# Autodesk Inventor assembly: 3組合1
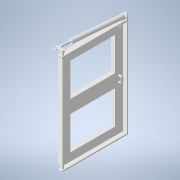
[picture p0: Inventor's stored thumbnail of the model, 180x180]
Saved by Autodesk Inventor 2020 (Build 240168000, 168)
## iProperties
Created: 2021-04-09
Part Number: 3組合1
Document SubType Name: Assembly
Designer: Sugar
Author: Sugar
## Documents named in this file (9)
- E:\github\cd2021\零件圖\stage2\3組合1.iam
- E:\github\cd2021\零件圖\stage2\3零件2.ipt
- E:\github\cd2021\零件圖\stage2\3零件3.ipt
- E:\github\cd2021\零件圖\stage2\3零件4.ipt
- E:\github\cd2021\零件圖\stage2\3零件5.ipt
- E:\github\cd2021\零件圖\stage2\3零件6.ipt
- E:\github\cd2021\零件圖\stage2\3零件7.ipt
- E:\github\cd2021\零件圖\stage2\3零件8.ipt
- E:\github\cd2021\零件圖\stage2\3零件10.ipt
## Components (8 placed, 8 different names)
1. 3零件5:1 — 插入:1, 貼合:4, 相切:1, 相切:2, 角度:2
2. 3零件6:1 — 貼合:1, 角度:1, 插入:5
3. 3零件7:2 — 插入:6
4. 3零件8:1 — 插入:1, 插入:2, 貼合:2
5. 3零件10:1 — 插入:2
6. 3零件2:1 — 插入:4, 插入:5, 插入:6, 相切:2
7. 3零件3:1 — 插入:3, 插入:4, 角度:1, 角度:2
8. 3零件4:1 — 插入:3, 貼合:4, 相切:1
## Relationships (14: Insert 6, Mate 4, Tangent 2, Angle 2)
- 插入:1 [Insert]: 3零件5:1 ↔ 3零件8:1
- 插入:2 [Insert]: 3零件8:1 ↔ 3零件10:1
- 貼合:1 [Mate]: 3零件6:1
- 貼合:2 [Mate]: 3零件8:1
- 貼合:3 [Mate]
- 插入:3 [Insert]: 3零件3:1 ↔ 3零件4:1
- 貼合:4 [Mate]: 3零件5:1 ↔ 3零件4:1
- 相切:1 [Tangent]: 3零件5:1 ↔ 3零件4:1
- 插入:4 [Insert]: 3零件2:1 ↔ 3零件3:1
- 角度:1 [Angle] (90 deg): 3零件6:1 ↔ 3零件3:1
- 插入:5 [Insert]: 3零件6:1 ↔ 3零件2:1
- 插入:6 [Insert]: 3零件7:2 ↔ 3零件2:1
- 相切:2 [Tangent]: 3零件5:1 ↔ 3零件2:1
- 角度:2 [Angle] (90 deg): 3零件5:1 ↔ 3零件3:1
